# Autodesk Inventor assembly: BackMountAssembly_SimplfiedVersion_MIR
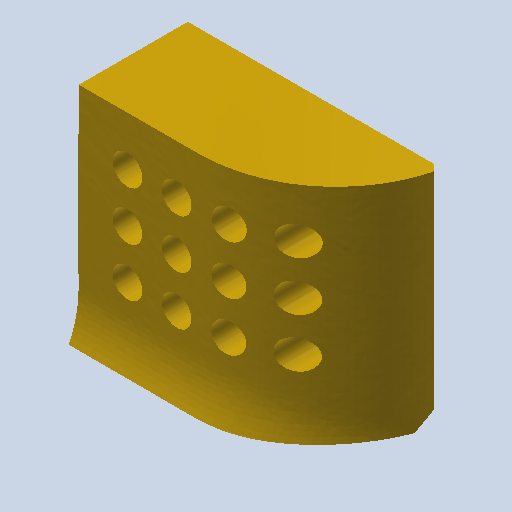
[picture p0: Inventor's stored thumbnail of the model, 512x512]
Saved by Autodesk Inventor 2022 (Build 260153000, 153)
## iProperties
Created: 2019-05-05
Part Number: BackMountAssembly_SimplfiedVersion_MIR
Document SubType Name: Assembly
Designer: CASE-SMALL2
Author: lgnds
## Documents named in this file (2)
- C:\Users\lgnds\Documents\GitHub\MARV-Hardware-Mechanical\InventorProjects\FMS - Front Mounting System\FästenFörRam\BackMountAssembly_SimplfiedVersion_MIR.iam
- C:\Users\lgnds\Documents\GitHub\MARV-Hardware-Mechanical\InventorProjects\FMS - Front Mounting System\FästenFörRam\BakV4_SimplifiedVersionV2_MIR.ipt
## Components (1 placed, 1 different names)
1. BakV4_SimplifiedVersionV2_MIR:1 — Flush:2, Flush:1, Mate:1
## Relationships (3: Mate 2, Flush 1)
- Flush:2 [Mate] (-45 mm): BakV4_SimplifiedVersionV2_MIR:1
- Flush:1 (58 mm): BakV4_SimplifiedVersionV2_MIR:1
- Mate:1 (183 mm): BakV4_SimplifiedVersionV2_MIR:1
